# Autodesk Inventor assembly: ballhand
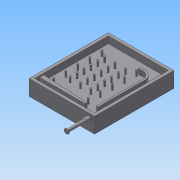
[picture p0: Inventor's stored thumbnail of the model, 180x180]
Saved by Autodesk Inventor 2017 (Build 210142000, 142)
## iProperties
Created: 2018-01-03
Part Number: ballhand
Document SubType Name: Assembly
Designer: user
Author: user
## Documents named in this file (3)
- F:\test\ball\ballhand.iam
- F:\test\ball\ball.ipt
- F:\test\ball\hand.ipt
## Components (2 placed, 2 different names)
1. ball:1 — 貼合:1, 齊平:1
2. hand:1 — 貼合:1, 齊平:1
## Relationships (2: Mate 1, Flush 1)
- 貼合:1 [Mate]: ball:1 ↔ hand:1
- 齊平:1 [Flush] (-2 mm): ball:1 ↔ hand:1
